# Autodesk Inventor assembly: BodyHipSupport
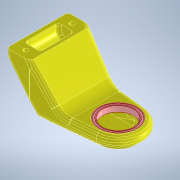
[picture p0: Inventor's stored thumbnail of the model, 180x180]
Saved by Autodesk Inventor 2022.2 (Build 262287000, 287)
## iProperties
Created: 2022-01-14
Part Number: BodyHipSupport
Document SubType Name: Assembly
Designer: Jochen
Author: Jochen
## Documents named in this file (3)
- D:\Projects\Chewbacca\CAD\Body\BodyHipSupport.iam
- D:\Projects\Chewbacca\CAD\Body\BodyHipSupport.ipt
- D:\Projects\Chewbacca\CAD\Common\Bearing\bearing_25_20_4_sbn_ET25202ZVA.ipt
## Components (2 placed, 2 different names)
1. BodyHipSupport:1 — Mate:1, Mate:2
2. bearing_25_20_4_sbn_ET25202ZVA:1 — Mate:1, Mate:2
## Relationships (2: Mate 2)
- Mate:1: BodyHipSupport:1 ↔ bearing_25_20_4_sbn_ET25202ZVA:1
- Mate:2: BodyHipSupport:1 ↔ bearing_25_20_4_sbn_ET25202ZVA:1
